# Autodesk Inventor assembly: Flashlight
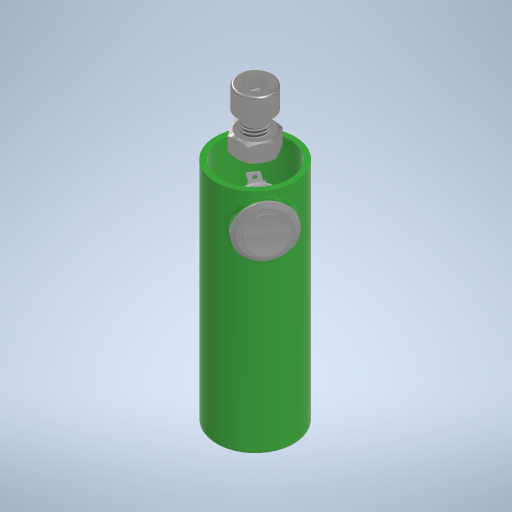
[picture p0: Inventor's stored thumbnail of the model, 512x512]
Saved by Autodesk Inventor 2024.2 (Build 282272000, 272)
## iProperties
Created: 2025-04-09
Part Number: Flashlight
Document SubType Name: Assembly
Designer: Svend
Author: Svend
## Documents named in this file (7)
- C:\Semesterprojekt\semesterproject_4_6\Inventor\Flashlight.iam
- C:\Semesterprojekt\semesterproject_4_6\Inventor\Flash_light.ipt
- C:\Users\Svend\OneDrive - Syddansk Universitet\2 semester\Semesterprojekt i autonome robotter\HG37-300-AB-00\3D\Battery_Holder_3AA_V1.ipt
- C:\Semesterprojekt\semesterproject_4_6\Inventor\161130345-9-xb-rs601c-1020011bb-zp\xb-rs601c-1020011bb-zp.iam
- C:\Users\Svend\Documents\Inventor\Content Center Files\R2024\en-US\ISO 4762(1)\DIN EN ISO 4762 - M10 x 16.ipt
- C:\Users\Svend\Documents\Inventor\Content Center Files\R2024\en-US\ISO 4032(1)\ISO 4032 - M10DIN EN.ipt
- C:\Semesterprojekt\semesterproject_4_6\Inventor\fleshlight_pcb\fleshlight_pcb.iam
## Components (6 placed, 6 different names)
1. Flash_light:1 — Mate:1, Mate:2, Mate:3, Mate:4, Mate:5, Mate:6, Mate:7, Mate:8, Mate:9
2. Battery_Holder_3AA_V1:1 — Mate:1, Mate:2
3. xb-rs601c-1020011bb-zp:1 [sub-assembly] — Mate:3, Mate:4, Mate:5
4. DIN EN ISO 4762 M10 x 16:1 — Cylindrical:1, Mate:6, Mate:7
5. DIN EN 24032 M10:1 — Cylindrical:1
6. fleshlight_pcb:1 [sub-assembly]
## Relationships (10: Mate 9, CylindricalJoint 1)
- Mate:1: Flash_light:1 ↔ Battery_Holder_3AA_V1:1
- Mate:2: Flash_light:1 ↔ Battery_Holder_3AA_V1:1
- Mate:3 (0.2 mm): Flash_light:1 ↔ xb-rs601c-1020011bb-zp:1
- Mate:4: Flash_light:1 ↔ xb-rs601c-1020011bb-zp:1
- Mate:5: Flash_light:1 ↔ xb-rs601c-1020011bb-zp:1
- Cylindrical:1: DIN EN ISO 4762 M10 x 16:1 ↔ DIN EN 24032 M10:1
- Mate:6: Flash_light:1 ↔ DIN EN ISO 4762 M10 x 16:1
- Mate:7 (20 mm): Flash_light:1 ↔ DIN EN ISO 4762 M10 x 16:1
- Mate:8: Flash_light:1
- Mate:9: Flash_light:1
